# Autodesk Inventor assembly: Full Assembly
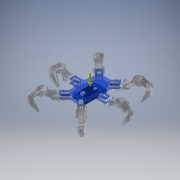
[picture p0: Inventor's stored thumbnail of the model, 180x180]
Saved by Autodesk Inventor 2016 (Build 200138000, 138)
## iProperties
Created: 2016-05-22
Part Number: Full Assembly
Document SubType Name: Assembly
Designer: Jacob
Author: Jacob
## Documents named in this file (10)
- H:\CAD\Hexapod\Full Assembly.iam
- H:\CAD\Hexapod\Servo Bracket 2.ipt
- H:\CAD\Hexapod\Servo Bracket 3.ipt
- H:\CAD\Hexapod\Servo Bracket.ipt
- H:\CAD\Hexapod\turnigy-tgy-s901d-digital-servo-1.snapshot.5 (1)\S901D.iam
- H:\CAD\Hexapod\Upper Chassis Plate.ipt
- H:\CAD\Hexapod\beagleboard-1.snapshot.3\Rough BeagleBone Black.ipt
- H:\CAD\Hexapod\Lower Chassis Plate.ipt
- H:\CAD\Hexapod\Battery.ipt
- H:\CAD\Hexapod\18mm Standoff.ipt
## Components (64 placed, 9 different names)
1. Servo Bracket 2:1 — Mate:46, Mate:47, Mate:48, Mate:67, Mate:68, Angle:5, Angle:6
2. Servo Bracket 3:1 — Mate:73, Mate:74, Mate:75, Angle:3
3. Servo Bracket:1 — Mate:25, Mate:26, Mate:35, Mate:36, Angle:4, Angle:5
4. Servo Bracket 2:2 — Mate:49, Mate:50, Mate:51, Mate:65, Mate:66, Angle:2, Angle:3
5. Servo Bracket 3:2 — Mate:85, Mate:86, Mate:87, Angle:12
6. Servo Bracket:2 — Mate:19, Mate:20, Mate:41, Mate:42, Angle:13, Angle:14
7. Servo Bracket 2:3 — Mate:58, Mate:59, Mate:60, Mate:69, Mate:70, Angle:8, Angle:9
8. Servo Bracket 3:3 — Mate:88, Mate:89, Mate:90, Angle:15
9. Servo Bracket:3 — Mate:29, Mate:30, Mate:39, Mate:40, Angle:10, Angle:11
10. Servo Bracket 2:4 — Mate:55, Mate:56, Mate:57, Mate:71, Mate:72, Angle:11, Angle:12
11. Servo Bracket 3:4 — Mate:82, Mate:83, Mate:84, Angle:9
12. Servo Bracket:4 — Mate:27, Mate:28, Mate:37, Mate:38, Angle:7, Angle:8
13. Servo Bracket 2:5 — Mate:52, Mate:53, Mate:54, Mate:61, Mate:62, Angle:14, Angle:15
14. Servo Bracket 3:5 — Mate:79, Mate:80, Mate:81, Angle:6
15. Servo Bracket:5 — Mate:23, Mate:24, Mate:33, Mate:34, Angle:1, Angle:2
16. Servo Bracket 2:6 — Mate:43, Mate:44, Mate:45, Mate:63, Mate:64, Angle:17, Angle:18
17. Servo Bracket 3:6 — Mate:76, Mate:77, Mate:78, Angle:18
18. Servo Bracket:6 — Mate:21, Mate:22, Mate:31, Mate:32, Angle:16, Angle:17
19. S901D:1 [sub-assembly] — Mate:65, Mate:66, Mate:73, Mate:74, Mate:75
20. S901D:2 [sub-assembly] — Mate:67, Mate:68, Mate:79, Mate:80, Mate:81
21. S901D:3 [sub-assembly] — Mate:61, Mate:62, Mate:88, Mate:89, Mate:90
22. S901D:4 [sub-assembly] — Mate:37, Mate:38, Mate:58, Mate:59, Mate:60
23. S901D:5 [sub-assembly] — Mate:33, Mate:34, Mate:49, Mate:50, Mate:51
24. S901D:6 [sub-assembly] — Mate:16, Mate:17, Mate:18, Mate:27, Mate:28
25. S901D:7 [sub-assembly] — Mate:13, Mate:14, Mate:15, Mate:25, Mate:26
26. S901D:8 [sub-assembly] — Mate:7, Mate:8, Mate:9, Mate:21, Mate:22
27. S901D:9 [sub-assembly] — Mate:1, Mate:2, Mate:3, Mate:29, Mate:30
28. S901D:10 [sub-assembly] — Mate:69, Mate:70, Mate:82, Mate:83, Mate:84
29. S901D:11 [sub-assembly] — Mate:71, Mate:72, Mate:85, Mate:86, Mate:87
30. S901D:12 [sub-assembly] — Mate:63, Mate:64, Mate:76, Mate:77, Mate:78
31. S901D:13 [sub-assembly] — Mate:41, Mate:42, Mate:52, Mate:53, Mate:54
32. S901D:14 [sub-assembly] — Mate:39, Mate:40, Mate:55, Mate:56, Mate:57
33. S901D:15 [sub-assembly] — Mate:35, Mate:36, Mate:46, Mate:47, Mate:48
34. S901D:16 [sub-assembly] — Mate:31, Mate:32, Mate:43, Mate:44, Mate:45
35. S901D:17 [sub-assembly] — Mate:10, Mate:11, Mate:12, Mate:23, Mate:24
36. S901D:18 [sub-assembly] — Mate:4, Mate:5, Mate:6, Mate:19, Mate:20
37. Upper Chassis Plate:1 — Mate:1, Mate:2, Mate:3, Mate:4, Mate:5, Mate:6, Mate:7, Mate:8, Mate:9, Mate:10, Mate:11, Mate:12, Mate:13, Mate:14, Mate:15, Mate:16, Mate:17, Mate:18, Angle:1, Angle:4, Angle:7, Angle:10, Angle:13, Angle:16, Angle:19, Mate:91, Flush:1, Flush:2, Mate:117, Mate:118, Mate:119, Mate:120, Mate:122, Mate:123, Mate:124, Mate:125, Mate:126, Mate:127, Mate:128, Mate:129, Mate:130, Mate:131, Mate:132, Mate:133, Mate:134, Mate:135, Mate:136, Mate:137, Mate:138, Mate:139, Mate:140
38. Rough BeagleBone Black:1 — Angle:19
39. Lower Chassis Plate:1 — Mate:91, Flush:1, Flush:2, Mate:92, Angle:20, Flush:3, Flush:4, Mate:93, Mate:94, Mate:95, Mate:96, Mate:97, Mate:98, Mate:99, Mate:100, Mate:101, Mate:102, Mate:103, Mate:104, Mate:105, Mate:106, Mate:107, Mate:108, Mate:109, Mate:110, Mate:111, Mate:112, Mate:113, Mate:114, Mate:115, Mate:116, Mate:121
40. Battery:1 — Mate:92, Angle:20, Flush:3, Flush:4
41. 18mm Standoff:1 — Mate:93, Mate:121
42. 18mm Standoff:2 — Mate:94, Mate:122
43. 18mm Standoff:3 — Mate:95, Mate:123
44. 18mm Standoff:4 — Mate:96, Mate:124
45. 18mm Standoff:5 — Mate:97, Mate:127
46. 18mm Standoff:6 — Mate:98, Mate:126
47. 18mm Standoff:7 — Mate:99, Mate:128
48. 18mm Standoff:8 — Mate:100, Mate:125
49. 18mm Standoff:9 — Mate:101, Mate:129
50. 18mm Standoff:10 — Mate:102, Mate:130
51. 18mm Standoff:11 — Mate:103, Mate:131
52. 18mm Standoff:12 — Mate:104, Mate:132
53. 18mm Standoff:13 — Mate:105, Mate:134
54. 18mm Standoff:14 — Mate:106, Mate:135
55. 18mm Standoff:15 — Mate:107, Mate:136
56. 18mm Standoff:16 — Mate:108, Mate:133
57. 18mm Standoff:17 — Mate:116, Mate:120
58. 18mm Standoff:18 — Mate:115, Mate:119
59. 18mm Standoff:19 — Mate:114, Mate:118
60. 18mm Standoff:20 — Mate:113, Mate:117
61. 18mm Standoff:21 — Mate:109, Mate:137
62. 18mm Standoff:22 — Mate:110, Mate:138
63. 18mm Standoff:23 — Mate:111, Mate:140
64. 18mm Standoff:24 — Mate:112, Mate:139
## Relationships (164: Mate 140, Angle 20, Flush 4)
- Mate:1: S901D:9 ↔ Upper Chassis Plate:1
- Mate:2: S901D:9 ↔ Upper Chassis Plate:1
- Mate:3: S901D:9 ↔ Upper Chassis Plate:1
- Mate:4: S901D:18 ↔ Upper Chassis Plate:1
- Mate:5: S901D:18 ↔ Upper Chassis Plate:1
- Mate:6: S901D:18 ↔ Upper Chassis Plate:1
- Mate:7: S901D:8 ↔ Upper Chassis Plate:1
- Mate:8: S901D:8 ↔ Upper Chassis Plate:1
- Mate:9: S901D:8 ↔ Upper Chassis Plate:1
- Mate:10: S901D:17 ↔ Upper Chassis Plate:1
- Mate:11: S901D:17 ↔ Upper Chassis Plate:1
- Mate:12: S901D:17 ↔ Upper Chassis Plate:1
- Mate:13: S901D:7 ↔ Upper Chassis Plate:1
- Mate:14: S901D:7 ↔ Upper Chassis Plate:1
- Mate:15: S901D:7 ↔ Upper Chassis Plate:1
- Mate:16: S901D:6 ↔ Upper Chassis Plate:1
- Mate:17: S901D:6 ↔ Upper Chassis Plate:1
- Mate:18: S901D:6 ↔ Upper Chassis Plate:1
- Mate:19: Servo Bracket:2 ↔ S901D:18
- Mate:20: Servo Bracket:2 ↔ S901D:18
- Mate:21: Servo Bracket:6 ↔ S901D:8
- Mate:22: Servo Bracket:6 ↔ S901D:8
- Mate:23: Servo Bracket:5 ↔ S901D:17
- Mate:24: Servo Bracket:5 ↔ S901D:17
- Mate:25: Servo Bracket:1 ↔ S901D:7
- Mate:26: Servo Bracket:1 ↔ S901D:7
- Mate:27: Servo Bracket:4 ↔ S901D:6
- Mate:28: Servo Bracket:4 ↔ S901D:6
- Mate:29: Servo Bracket:3 ↔ S901D:9
- Mate:30: Servo Bracket:3 ↔ S901D:9
- Mate:31: Servo Bracket:6 ↔ S901D:16
- Mate:32: Servo Bracket:6 ↔ S901D:16
- Mate:33: Servo Bracket:5 ↔ S901D:5
- Mate:34: Servo Bracket:5 ↔ S901D:5
- Mate:35: Servo Bracket:1 ↔ S901D:15
- Mate:36: Servo Bracket:1 ↔ S901D:15
- Mate:37: Servo Bracket:4 ↔ S901D:4
- Mate:38: Servo Bracket:4 ↔ S901D:4
- Mate:39: Servo Bracket:3 ↔ S901D:14
- Mate:40: Servo Bracket:3 ↔ S901D:14
- Mate:41: Servo Bracket:2 ↔ S901D:13
- Mate:42: Servo Bracket:2 ↔ S901D:13
- Mate:43: Servo Bracket 2:6 ↔ S901D:16
- Mate:44: Servo Bracket 2:6 ↔ S901D:16
- Mate:45: Servo Bracket 2:6 ↔ S901D:16
- Mate:46: Servo Bracket 2:1 ↔ S901D:15
- Mate:47: Servo Bracket 2:1 ↔ S901D:15
- Mate:48: Servo Bracket 2:1 ↔ S901D:15
- Mate:49: Servo Bracket 2:2 ↔ S901D:5
- Mate:50: Servo Bracket 2:2 ↔ S901D:5
- Mate:51: Servo Bracket 2:2 ↔ S901D:5
- Mate:52: Servo Bracket 2:5 ↔ S901D:13
- Mate:53: Servo Bracket 2:5 ↔ S901D:13
- Mate:54: Servo Bracket 2:5 ↔ S901D:13
- Mate:55: Servo Bracket 2:4 ↔ S901D:14
- Mate:56: Servo Bracket 2:4 ↔ S901D:14
- Mate:57: Servo Bracket 2:4 ↔ S901D:14
- Mate:58: Servo Bracket 2:3 ↔ S901D:4
- Mate:59: Servo Bracket 2:3 ↔ S901D:4
- Mate:60: Servo Bracket 2:3 ↔ S901D:4
- Mate:61: Servo Bracket 2:5 ↔ S901D:3
- Mate:62: Servo Bracket 2:5 ↔ S901D:3
- Mate:63: Servo Bracket 2:6 ↔ S901D:12
- Mate:64: Servo Bracket 2:6 ↔ S901D:12
- Mate:65: Servo Bracket 2:2 ↔ S901D:1
- Mate:66: Servo Bracket 2:2 ↔ S901D:1
- Mate:67: Servo Bracket 2:1 ↔ S901D:2
- Mate:68: Servo Bracket 2:1 ↔ S901D:2
- Mate:69: Servo Bracket 2:3 ↔ S901D:10
- Mate:70: Servo Bracket 2:3 ↔ S901D:10
- Mate:71: Servo Bracket 2:4 ↔ S901D:11
- Mate:72: Servo Bracket 2:4 ↔ S901D:11
- Mate:73: Servo Bracket 3:1 ↔ S901D:1
- Mate:74: Servo Bracket 3:1 ↔ S901D:1
- Mate:75: Servo Bracket 3:1 ↔ S901D:1
- Mate:76: Servo Bracket 3:6 ↔ S901D:12
- Mate:77: Servo Bracket 3:6 ↔ S901D:12
- Mate:78: Servo Bracket 3:6 ↔ S901D:12
- Mate:79: Servo Bracket 3:5 ↔ S901D:2
- Mate:80: Servo Bracket 3:5 ↔ S901D:2
- Mate:81: Servo Bracket 3:5 ↔ S901D:2
- Mate:82: Servo Bracket 3:4 ↔ S901D:10
- Mate:83: Servo Bracket 3:4 ↔ S901D:10
- Mate:84: Servo Bracket 3:4 ↔ S901D:10
- Mate:85: Servo Bracket 3:2 ↔ S901D:11
- Mate:86: Servo Bracket 3:2 ↔ S901D:11
- Mate:87: Servo Bracket 3:2 ↔ S901D:11
- Mate:88: Servo Bracket 3:3 ↔ S901D:3
- Mate:89: Servo Bracket 3:3 ↔ S901D:3
- Mate:90: Servo Bracket 3:3 ↔ S901D:3
- Angle:1 (0 deg): Servo Bracket:5 ↔ Upper Chassis Plate:1
- Angle:2 (30 deg): Servo Bracket 2:2 ↔ Servo Bracket:5
- Angle:3 (75 deg): Servo Bracket 3:1 ↔ Servo Bracket 2:2
- Angle:4 (0 deg): Servo Bracket:1 ↔ Upper Chassis Plate:1
- Angle:5 (30 deg): Servo Bracket 2:1 ↔ Servo Bracket:1
- Angle:6 (75 deg): Servo Bracket 2:1 ↔ Servo Bracket 3:5
- Angle:7 (0 deg): Servo Bracket:4 ↔ Upper Chassis Plate:1
- Angle:8 (30 deg): Servo Bracket 2:3 ↔ Servo Bracket:4
- Angle:9 (75 deg): Servo Bracket 2:3 ↔ Servo Bracket 3:4
- Angle:10 (0 deg): Servo Bracket:3 ↔ Upper Chassis Plate:1
- Angle:11 (30 deg): Servo Bracket:3 ↔ Servo Bracket 2:4
- Angle:12 (75 deg): Servo Bracket 3:2 ↔ Servo Bracket 2:4
- Angle:13 (0 deg): Servo Bracket:2 ↔ Upper Chassis Plate:1
- Angle:14 (30 deg): Servo Bracket:2 ↔ Servo Bracket 2:5
- Angle:15 (75 deg): Servo Bracket 3:3 ↔ Servo Bracket 2:5
- Angle:16 (0 deg): Servo Bracket:6 ↔ Upper Chassis Plate:1
- Angle:17 (30 deg): Servo Bracket 2:6 ↔ Servo Bracket:6
- Angle:18 (75 deg): Servo Bracket 2:6 ↔ Servo Bracket 3:6
- Angle:19 (0 deg): Upper Chassis Plate:1 ↔ Rough BeagleBone Black:1
- Mate:91 (18 mm): Upper Chassis Plate:1 ↔ Lower Chassis Plate:1
- Flush:1: Upper Chassis Plate:1 ↔ Lower Chassis Plate:1
- Flush:2: Upper Chassis Plate:1 ↔ Lower Chassis Plate:1
- Mate:92: Lower Chassis Plate:1 ↔ Battery:1
- Angle:20 (0 deg): Lower Chassis Plate:1 ↔ Battery:1
- Flush:3 (-78.479 mm): Lower Chassis Plate:1 ↔ Battery:1
- Flush:4 (36.561 mm): Lower Chassis Plate:1 ↔ Battery:1
- Mate:93: Lower Chassis Plate:1 ↔ 18mm Standoff:1
- Mate:94: Lower Chassis Plate:1 ↔ 18mm Standoff:2
- Mate:95: Lower Chassis Plate:1 ↔ 18mm Standoff:3
- Mate:96: Lower Chassis Plate:1 ↔ 18mm Standoff:4
- Mate:97: Lower Chassis Plate:1 ↔ 18mm Standoff:5
- Mate:98: Lower Chassis Plate:1 ↔ 18mm Standoff:6
- Mate:99: Lower Chassis Plate:1 ↔ 18mm Standoff:7
- Mate:100: Lower Chassis Plate:1 ↔ 18mm Standoff:8
- Mate:101: Lower Chassis Plate:1 ↔ 18mm Standoff:9
- Mate:102: Lower Chassis Plate:1 ↔ 18mm Standoff:10
- Mate:103: Lower Chassis Plate:1 ↔ 18mm Standoff:11
- Mate:104: Lower Chassis Plate:1 ↔ 18mm Standoff:12
- Mate:105: Lower Chassis Plate:1 ↔ 18mm Standoff:13
- Mate:106: Lower Chassis Plate:1 ↔ 18mm Standoff:14
- Mate:107: Lower Chassis Plate:1 ↔ 18mm Standoff:15
- Mate:108: Lower Chassis Plate:1 ↔ 18mm Standoff:16
- Mate:109: Lower Chassis Plate:1 ↔ 18mm Standoff:21
- Mate:110: Lower Chassis Plate:1 ↔ 18mm Standoff:22
- Mate:111: Lower Chassis Plate:1 ↔ 18mm Standoff:23
- Mate:112: Lower Chassis Plate:1 ↔ 18mm Standoff:24
- Mate:113: Lower Chassis Plate:1 ↔ 18mm Standoff:20
- Mate:114: Lower Chassis Plate:1 ↔ 18mm Standoff:19
- Mate:115: Lower Chassis Plate:1 ↔ 18mm Standoff:18
- Mate:116: Lower Chassis Plate:1 ↔ 18mm Standoff:17
- Mate:117: Upper Chassis Plate:1 ↔ 18mm Standoff:20
- Mate:118: Upper Chassis Plate:1 ↔ 18mm Standoff:19
- Mate:119: Upper Chassis Plate:1 ↔ 18mm Standoff:18
- Mate:120: Upper Chassis Plate:1 ↔ 18mm Standoff:17
- Mate:121: Lower Chassis Plate:1 ↔ 18mm Standoff:1
- Mate:122: Upper Chassis Plate:1 ↔ 18mm Standoff:2
- Mate:123: Upper Chassis Plate:1 ↔ 18mm Standoff:3
- Mate:124: Upper Chassis Plate:1 ↔ 18mm Standoff:4
- Mate:125: Upper Chassis Plate:1 ↔ 18mm Standoff:8
- Mate:126: Upper Chassis Plate:1 ↔ 18mm Standoff:6
- Mate:127: Upper Chassis Plate:1 ↔ 18mm Standoff:5
- Mate:128: Upper Chassis Plate:1 ↔ 18mm Standoff:7
- Mate:129: Upper Chassis Plate:1 ↔ 18mm Standoff:9
- Mate:130: Upper Chassis Plate:1 ↔ 18mm Standoff:10
- Mate:131: Upper Chassis Plate:1 ↔ 18mm Standoff:11
- Mate:132: Upper Chassis Plate:1 ↔ 18mm Standoff:12
- Mate:133: Upper Chassis Plate:1 ↔ 18mm Standoff:16
- Mate:134: Upper Chassis Plate:1 ↔ 18mm Standoff:13
- Mate:135: Upper Chassis Plate:1 ↔ 18mm Standoff:14
- Mate:136: Upper Chassis Plate:1 ↔ 18mm Standoff:15
- Mate:137: Upper Chassis Plate:1 ↔ 18mm Standoff:21
- Mate:138: Upper Chassis Plate:1 ↔ 18mm Standoff:22
- Mate:139: Upper Chassis Plate:1 ↔ 18mm Standoff:24
- Mate:140: Upper Chassis Plate:1 ↔ 18mm Standoff:23
## Named parameters: sa_0 = -0, sa_1 = -500, sa_2 = 1e-13
note: some values were not read from the file. Shown as the stored number, unit unknown: "sa_0", "sa_1", "sa_2".
